# Autodesk Inventor assembly: bed-holder-pair
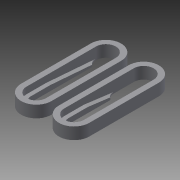
[picture p0: Inventor's stored thumbnail of the model, 180x180]
Saved by Autodesk Inventor 2015 (Build 190159000, 159)
## iProperties
Created: 2014-10-22
Part Number: bed-holder-pair
Document SubType Name: Assembly
Designer: caleb
Author: caleb
## Documents named in this file (3)
- C:\cygwin64\home\caleb\caleb-typea-settings\designs\simple-glass-bed\bed-holder-pair.iam
- C:\cygwin64\home\caleb\caleb-typea-settings\designs\simple-glass-bed\bed-holder.ipt
- C:\cygwin64\home\caleb\caleb-typea-settings\designs\simple-glass-bed\bed-holder-b.ipt
## Components (2 placed, 2 different names)
1. bed-holder:1 — Flush:1, Flush:2, Mate:1, Flush:3, Flush:4
2. bed-holder-b:1 — Flush:1, Flush:2
## Relationships (5: Flush 4, Mate 1)
- Flush:1: bed-holder:1 ↔ bed-holder-b:1
- Flush:2: bed-holder:1 ↔ bed-holder-b:1
- Mate:1: bed-holder:1
- Flush:3: bed-holder:1
- Flush:4: bed-holder:1
